# Autodesk Inventor assembly: Drive Tube Assem
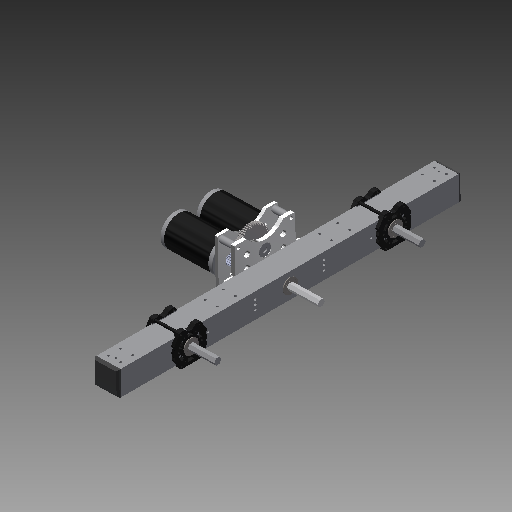
[picture p0: Inventor's stored thumbnail of the model, 512x512]
Saved by Autodesk Inventor 2018 (Build 220112000, 112)
## iProperties
Created: 2018-11-11
Part Number: Drive Tube Assem
Document SubType Name: Assembly
Designer: maste
Author: maste
## Documents named in this file (9)
- C:\Users\maste\OneDrive\Documents\GitHub\2019CAD\Summer Drivebase\Drive Tube Assem.iam
- C:\Users\maste\OneDrive\Documents\GitHub\2019CAD\Summer Drivebase\2x2 26in.ipt
- C:\Users\maste\OneDrive\Documents\GitHub\2019CAD\Summer Drivebase\Bearing Block Assem.iam
- C:\Users\maste\OneDrive\Documents\GitHub\2019CAD\Summer Drivebase\Gearbox Assem.iam
- C:\Users\maste\OneDrive\Documents\GitHub\2019CAD\Summer Drivebase\End Cap.ipt
- C:\Users\maste\OneDrive\Documents\GitHub\2019CAD\Summer Drivebase\217-3431-STEP.ipt
- C:\Users\maste\OneDrive\Documents\GitHub\2019CAD\Summer Drivebase\Middle Pulley Assembly.iam
- C:\Users\maste\OneDrive\Documents\GitHub\2019CAD\Summer Drivebase\Side Pulley Assembly Config 1.iam
- C:\Users\maste\OneDrive\Documents\GitHub\2019CAD\Summer Drivebase\Side Pulley Assembly Config 2.iam
## Components (11 placed, 8 different names)
1. 2x2 26in:1 — Mate:10, Mate:11, Rotation:1, Mate:12, Mate:13, Mate:14, Mate:15, Mate:16, Mate:17, Mate:18, Mate:19, Mate:20, Mate:21, Mate:22, Mate:23, Mate:24, Mate:25, Rotation:2, Mate:26, Mate:27, Rotation:3
2. Bearing Block Assem:1 [sub-assembly] — Mate:1, Mate:2, Mate:3, Mate:15, Mate:16, Mate:17
3. Bearing Block Assem:2 [sub-assembly] — Mate:4, Mate:5, Mate:6, Mate:12, Mate:13, Mate:14
4. Gearbox Assem:1 [sub-assembly] — Mate:7, Mate:8, Mate:9, Rotation:1
5. End Cap:1 — Mate:18, Mate:19, Mate:20
6. End Cap:2 — Mate:21, Mate:22, Mate:23
7. 217-3431-STEP:1 — Mate:26, Mate:27, Rotation:3
8. 217-3431-STEP:2 — Mate:24, Mate:25, Rotation:2
9. Middle Pulley Assembly:1 [sub-assembly] — Mate:7, Mate:8, Mate:9, Mate:10, Mate:11
10. Side Pulley Assembly Config 1:1 [sub-assembly] — Mate:1, Mate:2, Mate:3
11. Side Pulley Assembly Config 2:1 [sub-assembly] — Mate:4, Mate:5, Mate:6
## Relationships (30: Mate 27, RelateRotation 3)
- Mate:1: Bearing Block Assem:1 ↔ Side Pulley Assembly Config 1:1
- Mate:2: Bearing Block Assem:1 ↔ Side Pulley Assembly Config 1:1
- Mate:3: Bearing Block Assem:1 ↔ Side Pulley Assembly Config 1:1
- Mate:4: Bearing Block Assem:2 ↔ Side Pulley Assembly Config 2:1
- Mate:5: Bearing Block Assem:2 ↔ Side Pulley Assembly Config 2:1
- Mate:6: Bearing Block Assem:2 ↔ Side Pulley Assembly Config 2:1
- Mate:7: Gearbox Assem:1 ↔ Middle Pulley Assembly:1
- Mate:8: Gearbox Assem:1 ↔ Middle Pulley Assembly:1
- Mate:9: Gearbox Assem:1 ↔ Middle Pulley Assembly:1
- Mate:10: 2x2 26in:1 ↔ Middle Pulley Assembly:1
- Mate:11: 2x2 26in:1 ↔ Middle Pulley Assembly:1
- Rotation:1 [RelateRotation] (1 ul): 2x2 26in:1 ↔ Gearbox Assem:1
- Mate:12: 2x2 26in:1 ↔ Bearing Block Assem:2
- Mate:13: 2x2 26in:1 ↔ Bearing Block Assem:2
- Mate:14: 2x2 26in:1 ↔ Bearing Block Assem:2
- Mate:15: 2x2 26in:1 ↔ Bearing Block Assem:1
- Mate:16: 2x2 26in:1 ↔ Bearing Block Assem:1
- Mate:17: 2x2 26in:1 ↔ Bearing Block Assem:1
- Mate:18: 2x2 26in:1 ↔ End Cap:1
- Mate:19: 2x2 26in:1 ↔ End Cap:1
- Mate:20: 2x2 26in:1 ↔ End Cap:1
- Mate:21: 2x2 26in:1 ↔ End Cap:2
- Mate:22: 2x2 26in:1 ↔ End Cap:2
- Mate:23: 2x2 26in:1 ↔ End Cap:2
- Mate:24: 2x2 26in:1 ↔ 217-3431-STEP:2
- Mate:25: 2x2 26in:1 ↔ 217-3431-STEP:2
- Rotation:2 [RelateRotation] (1 ul): 2x2 26in:1 ↔ 217-3431-STEP:2
- Mate:26: 2x2 26in:1 ↔ 217-3431-STEP:1
- Mate:27: 2x2 26in:1 ↔ 217-3431-STEP:1
- Rotation:3 [RelateRotation] (1 ul): 2x2 26in:1 ↔ 217-3431-STEP:1
